# Autodesk Inventor assembly: GripperM120_2
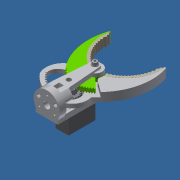
[picture p0: Inventor's stored thumbnail of the model, 180x180]
Saved by Autodesk Inventor 2016 (Build 200138000, 138)
## iProperties
Created: 2016-03-20
Part Number: GripperM120_2
Material: Generisch
Document SubType Name: Assembly
Designer: 4ndreas
Mass: 190.147 g
Surface Area: 586.131 cm^2
Volume: 124.392 cm^3
Density: 1.52862 g/cm^3
Parent: R6
Author: 4ndreas
## Documents named in this file (14)
- C:\Users\4ndreas\Documents\github\Mantis-Robot-Arm\MantisRobotArm\Workspace\Gripper V2\GripperM120_2.iam
- C:\Users\4ndreas\Documents\github\Mantis-Robot-Arm\MantisRobotArm\Workspace\Gripper V2\CloveM120\Konstruktions-Assistent\Stirnzahnrad12.ipt
- C:\Users\4ndreas\Documents\github\Mantis-Robot-Arm\MantisRobotArm\Workspace\Gripper V2\CloveM120\Konstruktions-Assistent\Stirnzahnrad13.ipt
- C:\Users\4ndreas\Documents\github\Mantis-Robot-Arm\MantisRobotArm\Workspace\_motors\servo.ipt
- C:\Users\4ndreas\Documents\github\Mantis-Robot-Arm\MantisRobotArm\Workspace\Gripper V2\ServoMount.ipt
- C:\Users\4ndreas\Documents\github\Mantis-Robot-Arm\MantisRobotArm\Libraries\Content Center Files\de-DE\DIN BEARING(1)\DIN 625 SKF - SKF 624.ipt
- C:\Users\4ndreas\Documents\github\Mantis-Robot-Arm\MantisRobotArm\Workspace\Gripper V2\Mount_B.ipt
- C:\Users\4ndreas\Documents\github\Mantis-Robot-Arm\MantisRobotArm\Workspace\Gripper V2\BearingGuide.ipt
- C:\Users\4ndreas\Documents\github\Mantis-Robot-Arm\MantisRobotArm\Libraries\Content Center Files\de-DE\DIN 912\DIN 912 - M4 x 0,7 x 40 x 20.ipt
- C:\Users\4ndreas\Documents\github\Mantis-Robot-Arm\MantisRobotArm\Libraries\Content Center Files\de-DE\DIN 125-1  A\DIN 125 - A 4,3.ipt
- C:\Users\4ndreas\Documents\github\Mantis-Robot-Arm\MantisRobotArm\Libraries\Content Center Files\de-DE\DIN 985\DIN 985 - M4.ipt
- C:\Users\4ndreas\Documents\github\Mantis-Robot-Arm\MantisRobotArm\Workspace\Gripper V2\Claw_3_l.ipt
- C:\Users\4ndreas\Documents\github\Mantis-Robot-Arm\MantisRobotArm\Workspace\Gripper V2\Claw_3_r.ipt
- C:\Users\4ndreas\Documents\github\Mantis-Robot-Arm\MantisRobotArm\Workspace\Gripper V2\Gear.ipt
## Components (17 placed, 11 different names)
1. Stirnzahnrad1:1 — Passend:3, Passend:4, Drehung:2, Drehung:3, Passend:13, Fluchtend:9
2. Stirnzahnrad1:2 — Passend:3, Passend:4, Passend:7, Drehung:1, Drehung:3
3. Stirnzahnrad2:3 — Passend:1, Passend:2, Fluchtend:6, Passend:8, Drehung:2, Passend:11, Passend:17, Fluchtend:9, Passend:22, Passend:23, Passend:24, Passend:26, Passend:28, Passend:30, Winkel:1
4. Stirnzahnrad2:4 — Passend:1, Passend:2, Passend:6, Drehung:1, Fluchtend:8, Passend:21, Passend:25, Passend:27, Passend:38
5. servo:1 — Passend:12, Passend:13, Passend:14, Fluchtend:7, Passend:15, Passend:16, Passend:37
6. ServoMount:1 — Fluchtend:7, Passend:15, Passend:16, Passend:35, Passend:36, Winkel:1
7. DIN 625 SKF SKF 624:1 — Passend:18, Passend:25
8. DIN 625 SKF SKF 624:2 — Passend:18, Passend:20, Passend:24
9. DIN 625 SKF SKF 624:3 — Passend:19, Passend:20, Passend:22, Passend:29
10. DIN 625 SKF SKF 624:4 — Passend:19, Passend:21, Passend:23, Fluchtend:10
11. Mount_B:1 — Fluchtend:11, Passend:33
12. BearingGuide:1 — Passend:26, Passend:27
13. BearingGuide:2 — Passend:28, Passend:29
14. DIN 912 - ersetzt durch DIN EN ISO 4762 M4 x 40:1 — Passend:30, Passend:31, Passend:32, Passend:34
15. DIN 125-1 A A 4,3:1 — Passend:31, Passend:32, Passend:33
16. DIN 985 - ersetzt durch DIN EN ISO 10511 M4:1 — Passend:34, Passend:35, Passend:36
17. Gear:1 — Passend:37, Passend:38
## Relationships (46: Mate 36, Flush 6, RelateRotation 3, Angle 1)
- Passend:1 [Mate]: Stirnzahnrad2:3 ↔ Stirnzahnrad2:4
- Passend:2 [Mate] (0.5 mm): Stirnzahnrad2:3 ↔ Stirnzahnrad2:4
- Passend:3 [Mate]: Stirnzahnrad1:1 ↔ Stirnzahnrad1:2
- Passend:4 [Mate]: Stirnzahnrad1:1 ↔ Stirnzahnrad1:2
- Fluchtend:6 [Flush]: Stirnzahnrad2:3
- Passend:6 [Mate]: Stirnzahnrad2:4
- Passend:7 [Mate]: Stirnzahnrad1:2
- Passend:8 [Mate]: Stirnzahnrad2:3
- Passend:9 [Mate] (39 mm)
- Drehung:1 [RelateRotation] (0.25 ul): Stirnzahnrad1:2 ↔ Stirnzahnrad2:4
- Drehung:2 [RelateRotation] (0.25 ul): Stirnzahnrad1:1 ↔ Stirnzahnrad2:3
- Drehung:3 [RelateRotation] (1 ul): Stirnzahnrad1:1 ↔ Stirnzahnrad1:2
- Passend:11 [Mate]: Stirnzahnrad2:3
- Passend:12 [Mate]: servo:1
- Passend:13 [Mate] (2 mm): Stirnzahnrad1:1 ↔ servo:1
- Passend:14 [Mate]: servo:1
- Fluchtend:7 [Flush]: servo:1 ↔ ServoMount:1
- Passend:15 [Mate]: servo:1 ↔ ServoMount:1
- Passend:16 [Mate]: servo:1 ↔ ServoMount:1
- Passend:17 [Mate]: Stirnzahnrad2:3
- Fluchtend:8 [Flush]: Stirnzahnrad2:4
- Fluchtend:9 [Flush]: Stirnzahnrad1:1 ↔ Stirnzahnrad2:3
- Passend:18 [Mate]: DIN 625 SKF SKF 624:1 ↔ DIN 625 SKF SKF 624:2
- Passend:19 [Mate]: DIN 625 SKF SKF 624:3 ↔ DIN 625 SKF SKF 624:4
- Passend:20 [Mate]: DIN 625 SKF SKF 624:2 ↔ DIN 625 SKF SKF 624:3
- Passend:21 [Mate]: Stirnzahnrad2:4 ↔ DIN 625 SKF SKF 624:4
- Passend:22 [Mate]: Stirnzahnrad2:3 ↔ DIN 625 SKF SKF 624:3
- Passend:23 [Mate]: Stirnzahnrad2:3 ↔ DIN 625 SKF SKF 624:4
- Passend:24 [Mate]: Stirnzahnrad2:3 ↔ DIN 625 SKF SKF 624:2
- Passend:25 [Mate]: Stirnzahnrad2:4 ↔ DIN 625 SKF SKF 624:1
- Fluchtend:10 [Flush] (1 mm): DIN 625 SKF SKF 624:4
- Fluchtend:11 [Flush]: Mount_B:1
- Passend:26 [Mate]: Stirnzahnrad2:3 ↔ BearingGuide:1
- Passend:27 [Mate]: Stirnzahnrad2:4 ↔ BearingGuide:1
- Passend:28 [Mate]: Stirnzahnrad2:3 ↔ BearingGuide:2
- Passend:29 [Mate]: DIN 625 SKF SKF 624:3 ↔ BearingGuide:2
- Passend:30 [Mate]: Stirnzahnrad2:3 ↔ DIN 912 - ersetzt durch DIN EN ISO 4762 M4 x 40:1
- Passend:31 [Mate]: DIN 912 - ersetzt durch DIN EN ISO 4762 M4 x 40:1 ↔ DIN 125-1 A A 4,3:1
- Passend:32 [Mate]: DIN 912 - ersetzt durch DIN EN ISO 4762 M4 x 40:1 ↔ DIN 125-1 A A 4,3:1
- Passend:33 [Mate]: Mount_B:1 ↔ DIN 125-1 A A 4,3:1
- Passend:34 [Mate]: DIN 912 - ersetzt durch DIN EN ISO 4762 M4 x 40:1 ↔ DIN 985 - ersetzt durch DIN EN ISO 10511 M4:1
- Passend:35 [Mate]: ServoMount:1 ↔ DIN 985 - ersetzt durch DIN EN ISO 10511 M4:1
- Passend:36 [Mate]: ServoMount:1 ↔ DIN 985 - ersetzt durch DIN EN ISO 10511 M4:1
- Passend:37 [Mate]: servo:1 ↔ Gear:1
- Passend:38 [Mate] (0.5 mm): Stirnzahnrad2:4 ↔ Gear:1
- Winkel:1 [Angle] (0 deg): Stirnzahnrad2:3 ↔ ServoMount:1
